# Autodesk Inventor assembly: Support
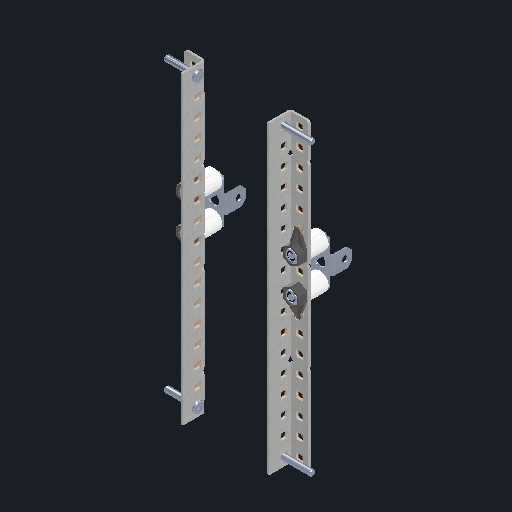
[picture p0: Inventor's stored thumbnail of the model, 512x512]
Saved by Autodesk Inventor 2025 (Build 290162000, 162)
## iProperties
Created: 2024-12-29
Part Number: Support
Document SubType Name: Assembly
Designer: Averey Ku
Author: Averey Ku
## Documents named in this file (8)
- D:\VEX\High Stakes\CAD\V4\Conveyer\Support.iam
- D:\VEX\High Stakes\CAD\ROBOPROS-CAD-Inventor\Structure\C Channel\Aluminum 1x3x1 Half Thick Cut\Alu C Half Thick 1x3x1x17.ipt
- D:\VEX\High Stakes\CAD\ROBOPROS-CAD-Inventor\Motion\Spacers\Spacer Nylon .500 OD\NSpacer White .500 OD x .500.ipt
- D:\VEX\High Stakes\CAD\ROBOPROS-CAD-Inventor\Motion\Spacers\Spacer Nylon .500 OD.ipt
- D:\VEX\High Stakes\CAD\ROBOPROS-CAD-Inventor\Motion\Pneumatics\Cylinder Rod Pivot.ipt
- D:\VEX\High Stakes\CAD\ROBOPROS-CAD-Inventor\Structure\Hardware\Screw Steel - Star\SScrew Star Smooth .875.ipt
- D:\VEX\High Stakes\CAD\ROBOPROS-CAD-Inventor\Structure\Hardware\Screw Steel - Star.ipt
- D:\VEX\High Stakes\CAD\ROBOPROS-CAD-Inventor\Structure\1-Post Hex Nut Retainer With Hardware.iam
## Components (20 placed, 5 different names)
1. Alu C Half Thick 1x3x1x17:1 — Mate:1, Mate:2, Mate:3, Insert:7, Mate:4, Mate:5, Mate:6, Insert:8, Insert:9
2. NSpacer White .500 OD x .500:1 — Insert:2, Insert:5, Mate:4
3. NSpacer White .500 OD x .500:2 — Insert:1, Insert:6, Insert:7
4. Cylinder Rod Pivot:1 — Insert:1, Insert:2, Insert:3, Insert:4
5. SScrew Star Smooth .875:1 — Insert:4
6. SScrew Star Smooth .875:2 — Insert:3
7. 1-Post Hex Nut Retainer With Hardware:1 [sub-assembly] — Insert:6, Mate:6
8. 1-Post Hex Nut Retainer With Hardware:2 [sub-assembly] — Insert:5, Mate:5
9. SScrew Star Smooth .875:3 — Insert:8
10. SScrew Star Smooth .875:4 — Insert:9
11. Alu C Half Thick 1x3x1x17:2 — Mate:7, Mate:8, Flush:1, Mate:9, Insert:10, Mate:10, Mate:11, Insert:17, Insert:18
12. NSpacer White .500 OD x .500:3 — Mate:9, Insert:11, Insert:16
13. NSpacer White .500 OD x .500:4 — Insert:10, Insert:12, Insert:15
14. Cylinder Rod Pivot:2 — Insert:11, Insert:12, Insert:13, Insert:14
15. SScrew Star Smooth .875:5 — Insert:13
16. SScrew Star Smooth .875:6 — Insert:14
17. 1-Post Hex Nut Retainer With Hardware:3 [sub-assembly] — Mate:10, Insert:15
18. 1-Post Hex Nut Retainer With Hardware:4 [sub-assembly] — Mate:11, Insert:16
19. SScrew Star Smooth .875:7 — Insert:17
20. SScrew Star Smooth .875:8 — Insert:18
## Relationships (30: Insert 18, Mate 11, Flush 1)
- Mate:1 (29.7434 mm): Alu C Half Thick 1x3x1x17:1
- Mate:2: Alu C Half Thick 1x3x1x17:1
- Mate:3 (-107.95 mm): Alu C Half Thick 1x3x1x17:1
- Insert:1: NSpacer White .500 OD x .500:2 ↔ Cylinder Rod Pivot:1
- Insert:2: NSpacer White .500 OD x .500:1 ↔ Cylinder Rod Pivot:1
- Insert:3: Cylinder Rod Pivot:1 ↔ SScrew Star Smooth .875:2
- Insert:4: Cylinder Rod Pivot:1 ↔ SScrew Star Smooth .875:1
- Insert:5 (1.5875 mm): NSpacer White .500 OD x .500:1 ↔ 1-Post Hex Nut Retainer With Hardware:2
- Insert:6 (1.5875 mm): NSpacer White .500 OD x .500:2 ↔ 1-Post Hex Nut Retainer With Hardware:1
- Insert:7: Alu C Half Thick 1x3x1x17:1 ↔ NSpacer White .500 OD x .500:2
- Mate:4: Alu C Half Thick 1x3x1x17:1 ↔ NSpacer White .500 OD x .500:1
- Mate:5: Alu C Half Thick 1x3x1x17:1 ↔ 1-Post Hex Nut Retainer With Hardware:2
- Mate:6: Alu C Half Thick 1x3x1x17:1 ↔ 1-Post Hex Nut Retainer With Hardware:1
- Insert:8: Alu C Half Thick 1x3x1x17:1 ↔ SScrew Star Smooth .875:3
- Insert:9: Alu C Half Thick 1x3x1x17:1 ↔ SScrew Star Smooth .875:4
- Mate:7 (-107.95 mm): Alu C Half Thick 1x3x1x17:2
- Mate:8: Alu C Half Thick 1x3x1x17:2
- Flush:1 (29.7434 mm): Alu C Half Thick 1x3x1x17:2
- Mate:9: Alu C Half Thick 1x3x1x17:2 ↔ NSpacer White .500 OD x .500:3
- Insert:10: Alu C Half Thick 1x3x1x17:2 ↔ NSpacer White .500 OD x .500:4
- Insert:11: NSpacer White .500 OD x .500:3 ↔ Cylinder Rod Pivot:2
- Insert:12: NSpacer White .500 OD x .500:4 ↔ Cylinder Rod Pivot:2
- Insert:13: Cylinder Rod Pivot:2 ↔ SScrew Star Smooth .875:5
- Insert:14: Cylinder Rod Pivot:2 ↔ SScrew Star Smooth .875:6
- Mate:10: Alu C Half Thick 1x3x1x17:2 ↔ 1-Post Hex Nut Retainer With Hardware:3
- Insert:15 (1.5875 mm): NSpacer White .500 OD x .500:4 ↔ 1-Post Hex Nut Retainer With Hardware:3
- Mate:11: Alu C Half Thick 1x3x1x17:2 ↔ 1-Post Hex Nut Retainer With Hardware:4
- Insert:16 (1.5875 mm): NSpacer White .500 OD x .500:3 ↔ 1-Post Hex Nut Retainer With Hardware:4
- Insert:17: Alu C Half Thick 1x3x1x17:2 ↔ SScrew Star Smooth .875:7
- Insert:18: Alu C Half Thick 1x3x1x17:2 ↔ SScrew Star Smooth .875:8
